# Autodesk Inventor assembly: pc4t
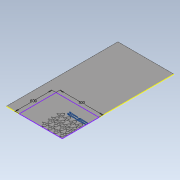
[picture p0: Inventor's stored thumbnail of the model, 180x180]
Saved by Autodesk Inventor 2020.3 (Build 243373000, 373)
## iProperties
Created: 2020-05-22
Part Number: pc4t
Document SubType Name: Assembly
Designer: aoyama
Author: aoyama
## Documents named in this file (4)
- C:\Users\aoyam\Desktop\SRDC_local\Inventor\二年機\Geminiβ\pc5t.iam
- C:\Users\aoyam\Desktop\SRDC_local\Inventor\二年機\PC板サイズ測定板.ipt
- C:\Users\aoyam\Desktop\SRDC_local\Inventor\二年機\Geminiβ\脚\ネジクランク\ヘッケン改.ipt
- C:\Users\aoyam\Desktop\SRDC_local\Inventor\二年機\Geminiβ\翼\ウィング.ipt
## Components (21 placed, 3 different names)
1. PC板サイズ測定板:1 — メイト:1, メイト:2, メイト:3, メイト:4, メイト:5, メイト:6, メイト:7, メイト:8, メイト:9, メイト:10, メイト:11, メイト:12, メイト:13, メイト:14, メイト:15, メイト:16, メイト:17, メイト:18, メイト:19, メイト:20
2. ヘッケン改:1 — メイト:6
3. ヘッケン改:2 — メイト:5
4. ヘッケン改:3 — メイト:4
5. ヘッケン改:4 — メイト:3
6. ヘッケン改:5 — メイト:2
7. ヘッケン改:6 — メイト:1
8. ヘッケン改:7 — メイト:7
9. ヘッケン改:8 — メイト:8
10. ヘッケン改:9 — メイト:9
11. ヘッケン改:10 — メイト:10
12. ヘッケン改:11 — メイト:11
13. ヘッケン改:12 — メイト:12
14. ヘッケン改:13 — メイト:13
15. ヘッケン改:14 — メイト:14
16. ヘッケン改:15 — メイト:15
17. ヘッケン改:16 — メイト:16
18. ウィング:1 — メイト:17
19. ウィング:2 — メイト:18
20. ウィング:3 — メイト:19
21. ウィング:4 — メイト:20
## Relationships (20: Mate 20)
- メイト:1 [Mate]: PC板サイズ測定板:1 ↔ ヘッケン改:6
- メイト:2 [Mate]: PC板サイズ測定板:1 ↔ ヘッケン改:5
- メイト:3 [Mate]: PC板サイズ測定板:1 ↔ ヘッケン改:4
- メイト:4 [Mate]: PC板サイズ測定板:1 ↔ ヘッケン改:3
- メイト:5 [Mate]: PC板サイズ測定板:1 ↔ ヘッケン改:2
- メイト:6 [Mate]: PC板サイズ測定板:1 ↔ ヘッケン改:1
- メイト:7 [Mate]: PC板サイズ測定板:1 ↔ ヘッケン改:7
- メイト:8 [Mate]: PC板サイズ測定板:1 ↔ ヘッケン改:8
- メイト:9 [Mate]: PC板サイズ測定板:1 ↔ ヘッケン改:9
- メイト:10 [Mate]: PC板サイズ測定板:1 ↔ ヘッケン改:10
- メイト:11 [Mate]: PC板サイズ測定板:1 ↔ ヘッケン改:11
- メイト:12 [Mate]: PC板サイズ測定板:1 ↔ ヘッケン改:12
- メイト:13 [Mate]: PC板サイズ測定板:1 ↔ ヘッケン改:13
- メイト:14 [Mate]: PC板サイズ測定板:1 ↔ ヘッケン改:14
- メイト:15 [Mate]: PC板サイズ測定板:1 ↔ ヘッケン改:15
- メイト:16 [Mate]: PC板サイズ測定板:1 ↔ ヘッケン改:16
- メイト:17 [Mate]: PC板サイズ測定板:1 ↔ ウィング:1
- メイト:18 [Mate]: PC板サイズ測定板:1 ↔ ウィング:2
- メイト:19 [Mate]: PC板サイズ測定板:1 ↔ ウィング:3
- メイト:20 [Mate]: PC板サイズ測定板:1 ↔ ウィング:4
